# Autodesk Inventor assembly: Completo
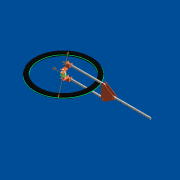
[picture p0: Inventor's stored thumbnail of the model, 180x180]
Saved by Autodesk Inventor 2016 (Build 200138000, 138)
## iProperties
Created: 2017-05-13
Part Number: Completo
Document SubType Name: Assembly
Designer: Gian
Author: Gian
## Documents named in this file (5)
- C:\Users\Gian\Desktop\Pedalazo\002_Diseño\Version_001\Completo.iam
- C:\Users\Gian\Desktop\Pedalazo\002_Diseño\Version_001\Conexion_rueda.ipt
- C:\Users\Gian\Desktop\Pedalazo\002_Diseño\Version_001\Rueda.ipt
- C:\Users\Gian\Desktop\Pedalazo\002_Diseño\Version_001\Tubo_conexion.ipt
- C:\Users\Gian\Desktop\Pedalazo\002_Diseño\Version_001\Conexion_eje.ipt
## Components (8 placed, 4 different names)
1. Conexion_rueda:1 — Flush:1, Flush:2, Insert:2
2. Conexion_rueda:2 — Flush:1, Flush:2, Flush:3, Insert:1
3. Rueda:1 — Flush:3
4. Tubo_conexion:1 — Insert:1
5. Tubo_conexion:2 — Insert:2
6. Conexion_eje:1
7. Conexion_eje:2
8. Tubo_conexion:3
## Relationships (5: Flush 3, Insert 2)
- Flush:1: Conexion_rueda:1 ↔ Conexion_rueda:2
- Flush:2: Conexion_rueda:1 ↔ Conexion_rueda:2
- Flush:3: Conexion_rueda:2 ↔ Rueda:1
- Insert:1: Conexion_rueda:2 ↔ Tubo_conexion:1
- Insert:2: Conexion_rueda:1 ↔ Tubo_conexion:2
